# Autodesk Inventor assembly: ASM_Micron_ASAP_Merge
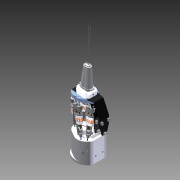
[picture p0: Inventor's stored thumbnail of the model, 180x180]
Saved by Autodesk Inventor 2011 SP2 (Build 150309200, 309)
## iProperties
Created: 2011-10-07
Part Number: ASM_Micron_ASAP_Merge
Document SubType Name: Assembly
Designer: sungwook
Author: sungwook
## Documents named in this file (20)
- C:\Users\sungwook\Documents\Inventor\Micron20\Assembly\Motion_Merge\ASM_Micron_ASAP_Merge1.iam
- C:\Users\sungwook\Documents\Inventor\Micron20\Assembly\Motion_Merge\ASM_Micron_ASAP_Indep0.iam
- C:\Users\sungwook\Documents\Inventor\Micron20\Assembly\Motion_Merge\ASM_Micron_ASAP_Indep10.iam
- C:\Users\sungwook\Documents\Inventor\Micron20\Assembly\Motion_Merge\ASM_Micron_ASAP_Indep20.iam
- C:\Users\sungwook\Documents\Inventor\Micron20\Assembly\Motion_Merge\ASM_Micron_ASAP_Indep30.iam
- C:\Users\sungwook\Documents\Inventor\Micron20\Assembly\Motion_Merge\ASM_Micron_ASAP_Indep40.iam
- C:\Users\sungwook\Documents\Inventor\Micron20\Assembly\Motion_Merge\ASM_Micron_ASAP_Indep50.iam
- C:\Users\sungwook\Documents\Inventor\Micron20\Assembly\Motion_Merge\ASM_Micron_ASAP_Indep60.iam
- C:\Users\sungwook\Documents\Inventor\Micron20\Assembly\Motion_Merge\ASM_Micron_ASAP_Indep70.iam
- C:\Users\sungwook\Documents\Inventor\Micron20\Assembly\Motion_Merge\ASM_Micron_ASAP_Indep80.iam
- C:\Users\sungwook\Documents\Inventor\Micron20\Assembly\Motion_Merge\ASM_Micron_ASAP_Indep90.iam
- C:\Users\sungwook\Documents\Inventor\Micron20\Assembly\Motion_Merge\ASM_Micron_ASAP_Indep100.iam
- C:\Users\sungwook\Documents\Inventor\Micron20\Assembly\Motion_Merge\ASM_Micron_ASAP_Indep110.iam
- C:\Users\sungwook\Documents\Inventor\Micron20\Assembly\Motion_Merge\ASM_Micron_ASAP_Indep120.iam
- C:\Users\sungwook\Documents\Inventor\Micron20\Assembly\Motion_Merge\ASM_Micron_ASAP_Indep130.iam
- C:\Users\sungwook\Documents\Inventor\Micron20\Assembly\Motion_Merge\ASM_Micron_ASAP_Indep140.iam
- C:\Users\sungwook\Documents\Inventor\Micron17_Rev1\Parts\Case\Case2.ipt
- C:\Users\sungwook\Documents\Inventor\Micron17_Rev1\Parts\ASAP\ASAP_Top_Fixture_Handle.ipt
- C:\Users\sungwook\Documents\Inventor\Micron17_Rev1\Parts\Case\Case4_Short.ipt
- C:\Users\sungwook\Documents\Inventor\Micron17_Rev1\Parts\Case\Case4_Short_Wall_Adj.ipt
## Components (19 placed, 19 different names)
1. (0,0,0) [sub-assembly] — Mate:1, Flush:1, Flush:2, Flush:3, Mate:2, Flush:4, Mate:3, Flush:5, Flush:6, Mate:4, Flush:7, Flush:8, Mate:5, Flush:9, Flush:10, Flush:11, Flush:12, Mate:6, Mate:7, Flush:13, Flush:14, Flush:16, Mate:9, Flush:17, Flush:18, Mate:10, Flush:19, Mate:11, Flush:20, Flush:21, Mate:15, Flush:22, Flush:23, Flush:24, Flush:25, Flush:26, Flush:27, Flush:28
2. (0,2,0) [sub-assembly] — Mate:1, Flush:1, Flush:2
3. pi/2,2,0 [sub-assembly] — Flush:3, Flush:4
4. pi,2,0 [sub-assembly] — Mate:3, Flush:5, Flush:6
5. -pi/2,2,0 [sub-assembly] — Mate:4, Flush:7, Flush:8
6. 0,0,-2 [sub-assembly] — Mate:5, Flush:9, Flush:10
7. 0,2,-2 [sub-assembly] — Flush:11, Flush:12, Mate:6
8. pi/2,2,-2 [sub-assembly] — Mate:11, Flush:20, Flush:21
9. pi,2,-2 [sub-assembly] — Mate:8, Flush:15, Flush:16
10. -pi/2,2,-2 [sub-assembly] — Mate:7, Flush:13, Flush:14, Mate:8, Flush:15, Flush:29
11. 0,0,2 [sub-assembly] — Mate:9, Flush:17, Flush:18
12. 0,2,2 [sub-assembly] — Mate:10, Flush:19, Flush:27, Flush:28
13. pi/2,2,2 [sub-assembly] — Mate:15, Flush:22
14. pi,2,2 [sub-assembly] — Mate:18, Flush:23, Flush:24
15. -pi/2,2,2 [sub-assembly] — Mate:19, Flush:25, Flush:26, Mate:22, Mate:23
16. Case2:1 — Mate:20, Angle:3
17. ASAP_Top_Fixture_Handle:1 — Mate:22, Mate:23, Flush:29
18. Case4_Short:1 — Mate:25, Flush:26
19. Case4_Short_Wall_Adj:1 — Mate:26, Flush:30
## Relationships (51: Flush 31, Mate 19, Angle 1)
- Mate:1: (0,0,0) ↔ (0,2,0)
- Flush:1: (0,0,0) ↔ (0,2,0)
- Flush:2: (0,0,0) ↔ (0,2,0)
- Flush:3: (0,0,0) ↔ pi/2,2,0
- Mate:2: (0,0,0)
- Flush:4: (0,0,0) ↔ pi/2,2,0
- Mate:3: (0,0,0) ↔ pi,2,0
- Flush:5: (0,0,0) ↔ pi,2,0
- Flush:6: (0,0,0) ↔ pi,2,0
- Mate:4: (0,0,0) ↔ -pi/2,2,0
- Flush:7: (0,0,0) ↔ -pi/2,2,0
- Flush:8: (0,0,0) ↔ -pi/2,2,0
- Mate:5: (0,0,0) ↔ 0,0,-2
- Flush:9: (0,0,0) ↔ 0,0,-2
- Flush:10: (0,0,0) ↔ 0,0,-2
- Flush:11: (0,0,0) ↔ 0,2,-2
- Flush:12: (0,0,0) ↔ 0,2,-2
- Mate:6: (0,0,0) ↔ 0,2,-2
- Mate:7: (0,0,0) ↔ -pi/2,2,-2
- Flush:13: (0,0,0) ↔ -pi/2,2,-2
- Flush:14: (0,0,0) ↔ -pi/2,2,-2
- Mate:8: pi,2,-2 ↔ -pi/2,2,-2
- Flush:15: pi,2,-2 ↔ -pi/2,2,-2
- Flush:16: (0,0,0) ↔ pi,2,-2
- Mate:9: (0,0,0) ↔ 0,0,2
- Flush:17: (0,0,0) ↔ 0,0,2
- Flush:18: (0,0,0) ↔ 0,0,2
- Mate:10: (0,0,0) ↔ 0,2,2
- Flush:19: (0,0,0) ↔ 0,2,2
- Mate:11: (0,0,0) ↔ pi/2,2,-2
- Flush:20: (0,0,0) ↔ pi/2,2,-2
- Flush:21: (0,0,0) ↔ pi/2,2,-2
- Mate:15: (0,0,0) ↔ pi/2,2,2
- Flush:22: (0,0,0) ↔ pi/2,2,2
- Mate:18: pi,2,2
- Flush:23: (0,0,0) ↔ pi,2,2
- Flush:24: (0,0,0) ↔ pi,2,2
- Mate:19: -pi/2,2,2
- Flush:25: (0,0,0) ↔ -pi/2,2,2
- Flush:26: (0,0,0) ↔ -pi/2,2,2
- Mate:20: Case2:1
- Angle:3 (-90 deg): Case2:1
- Flush:27: (0,0,0) ↔ 0,2,2
- Flush:28: (0,0,0) ↔ 0,2,2
- Mate:22: -pi/2,2,2 ↔ ASAP_Top_Fixture_Handle:1
- Mate:23: -pi/2,2,2 ↔ ASAP_Top_Fixture_Handle:1
- Flush:29 (-5 mm): -pi/2,2,-2 ↔ ASAP_Top_Fixture_Handle:1
- Mate:25: Case4_Short:1
- Flush:26: Case4_Short:1
- Mate:26: Case4_Short_Wall_Adj:1
- Flush:30: Case4_Short_Wall_Adj:1
